# Autodesk Inventor assembly: assy_mission_level_crossing
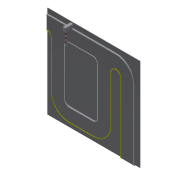
[picture p0: Inventor's stored thumbnail of the model, 180x180]
Saved by Autodesk Inventor 2018 (Build 220112000, 112)
## iProperties
Created: 2017-11-13
Part Number: assy_mission_level_crossing
Document SubType Name: Assembly
Designer: Platform
Author: Platform
## Documents named in this file (9)
- C:\Users\Platform\Desktop\autorace_track\track_model\autorace_rbizchallenge2017\assembled\assy_mission_level_crossing.iam
- C:\Users\Platform\Desktop\autorace_track\track_model\autorace_rbizchallenge2017\assembled\assy_lower_plates.iam
- C:\Users\Platform\Desktop\autorace_track\track_model\autorace_rbizchallenge2017\assembled\assy_straight.iam
- C:\Users\Platform\Desktop\autorace_track\track_model\autorace_rbizchallenge2017\assembled\assy_curved_left.iam
- C:\Users\Platform\Desktop\autorace_track\track_model\autorace_rbizchallenge2017\assembled\assy_three_way_intersection_left_open.iam
- C:\Users\Platform\Desktop\autorace_track\track_model\autorace_rbizchallenge2017\assembled\assy_curved_right.iam
- C:\Users\Platform\Desktop\autorace_track\track_model\autorace_rbizchallenge2017\assembled\assy_straight_both_white.iam
- C:\Users\Platform\Desktop\autorace_track\track_model\autorace_rbizchallenge2017\assembled\assy_three_way_intersection_left_closed.iam
- C:\Users\Platform\Desktop\autorace_track\track_model\autorace_rbizchallenge2017\parts\ipt\level.ipt
## Components (16 placed, 8 different names)
1. assy_lower_plates:1 [sub-assembly] — Mate:1, Flush:1, Flush:2, Mate:2, Mate:5, Mate:6, Mate:9, Mate:12, Mate:15, Mate:17, Mate:20, Mate:23, Mate:25, Mate:28, Mate:31, Mate:33, Mate:35
2. assy_straight:1 [sub-assembly] — Mate:1, Flush:1, Flush:2, Mate:3, Flush:3
3. assy_straight:2 [sub-assembly] — Mate:2, Mate:3, Flush:3, Mate:4, Flush:4
4. assy_straight:3 [sub-assembly] — Mate:4, Mate:5, Flush:4, Mate:7, Mate:8
5. assy_curved_left:1 [sub-assembly] — Mate:6, Mate:7, Mate:8, Mate:10, Mate:11
6. assy_three_way_intersection_left_open:1 [sub-assembly] — Mate:9, Mate:10, Mate:11, Mate:13, Mate:14, Mate:24, Flush:6
7. assy_straight:4 [sub-assembly] — Mate:12, Mate:13, Mate:14, Mate:16, Flush:5
8. assy_straight:5 [sub-assembly] — Mate:15, Mate:16, Flush:5, Mate:18, Mate:19
9. assy_curved_right:1 [sub-assembly] — Mate:17, Mate:18, Mate:19, Mate:21, Mate:22
10. assy_straight:6 [sub-assembly] — Mate:20, Mate:21, Mate:22, Mate:26, Mate:27
11. assy_straight_both_white:1 [sub-assembly] — Mate:23, Mate:24, Flush:6, Mate:34, Flush:8, Mate:36
12. assy_curved_right:2 [sub-assembly] — Mate:25, Mate:26, Mate:27, Mate:29, Mate:30
13. assy_straight:7 [sub-assembly] — Mate:28, Mate:29, Mate:30, Mate:32, Flush:7
14. assy_straight:8 [sub-assembly] — Mate:31, Mate:32, Flush:7
15. assy_three_way_intersection_left_closed:1 [sub-assembly] — Mate:33, Mate:34, Flush:8, Mate:37
16. level:1 — Mate:35, Mate:36, Mate:37
## Relationships (45: Mate 37, Flush 8)
- Mate:1: assy_lower_plates:1 ↔ assy_straight:1
- Flush:1 (100 mm): assy_lower_plates:1 ↔ assy_straight:1
- Flush:2: assy_lower_plates:1 ↔ assy_straight:1
- Mate:2: assy_lower_plates:1 ↔ assy_straight:2
- Mate:3: assy_straight:1 ↔ assy_straight:2
- Flush:3: assy_straight:1 ↔ assy_straight:2
- Mate:4: assy_straight:2 ↔ assy_straight:3
- Mate:5: assy_lower_plates:1 ↔ assy_straight:3
- Flush:4: assy_straight:2 ↔ assy_straight:3
- Mate:6: assy_lower_plates:1 ↔ assy_curved_left:1
- Mate:7: assy_straight:3 ↔ assy_curved_left:1
- Mate:8: assy_straight:3 ↔ assy_curved_left:1
- Mate:9: assy_lower_plates:1 ↔ assy_three_way_intersection_left_open:1
- Mate:10: assy_curved_left:1 ↔ assy_three_way_intersection_left_open:1
- Mate:11: assy_curved_left:1 ↔ assy_three_way_intersection_left_open:1
- Mate:12: assy_lower_plates:1 ↔ assy_straight:4
- Mate:13: assy_three_way_intersection_left_open:1 ↔ assy_straight:4
- Mate:14: assy_three_way_intersection_left_open:1 ↔ assy_straight:4
- Mate:15: assy_lower_plates:1 ↔ assy_straight:5
- Mate:16: assy_straight:4 ↔ assy_straight:5
- Flush:5: assy_straight:4 ↔ assy_straight:5
- Mate:17: assy_lower_plates:1 ↔ assy_curved_right:1
- Mate:18: assy_straight:5 ↔ assy_curved_right:1
- Mate:19: assy_straight:5 ↔ assy_curved_right:1
- Mate:20: assy_lower_plates:1 ↔ assy_straight:6
- Mate:21: assy_curved_right:1 ↔ assy_straight:6
- Mate:22: assy_curved_right:1 ↔ assy_straight:6
- Mate:23: assy_lower_plates:1 ↔ assy_straight_both_white:1
- Mate:24: assy_three_way_intersection_left_open:1 ↔ assy_straight_both_white:1
- Flush:6: assy_three_way_intersection_left_open:1 ↔ assy_straight_both_white:1
- Mate:25: assy_lower_plates:1 ↔ assy_curved_right:2
- Mate:26: assy_straight:6 ↔ assy_curved_right:2
- Mate:27: assy_straight:6 ↔ assy_curved_right:2
- Mate:28: assy_lower_plates:1 ↔ assy_straight:7
- Mate:29: assy_curved_right:2 ↔ assy_straight:7
- Mate:30: assy_curved_right:2 ↔ assy_straight:7
- Mate:31: assy_lower_plates:1 ↔ assy_straight:8
- Mate:32: assy_straight:7 ↔ assy_straight:8
- Flush:7: assy_straight:7 ↔ assy_straight:8
- Mate:33: assy_lower_plates:1 ↔ assy_three_way_intersection_left_closed:1
- Mate:34: assy_straight_both_white:1 ↔ assy_three_way_intersection_left_closed:1
- Flush:8: assy_straight_both_white:1 ↔ assy_three_way_intersection_left_closed:1
- Mate:35: assy_lower_plates:1 ↔ level:1
- Mate:36: assy_straight_both_white:1 ↔ level:1
- Mate:37: assy_three_way_intersection_left_closed:1 ↔ level:1
